# Autodesk Inventor assembly: HACKberry_v1_for_print_Hand_withCaseC
Saved by Autodesk Inventor 2016 (Build 200138000, 138)
## iProperties
Created: 2016-06-07
Part Number: HACKberry_v1_for_print_Hand_withCaseC
Material: 一般
Document SubType Name: Assembly
Designer: Yamaura
Author: Yamaura
## Documents named in this file (9)
- C:\Users\Yamaura\Documents\GitHub\HACKberry\HACKberry-hardware\3D\Inventor\Parts\HACKberry_v1_for_print_Hand_withCaseC.iam
- C:\Users\Yamaura\Documents\GitHub\HACKberry\HACKberry-hardware\3D\Inventor\Parts\HbBatteryCase01.ipt
- C:\Users\Yamaura\Documents\GitHub\HACKberry\HACKberry-hardware\3D\Inventor\Parts\HbMiddle-DistalPhalanx02.ipt
- C:\Users\Yamaura\Documents\GitHub\HACKberry\HACKberry-hardware\3D\Inventor\Parts\HbProximalPhalanx02.ipt
- C:\Users\Yamaura\Documents\GitHub\HACKberry\HACKberry-hardware\3D\Inventor\Parts\HbProximalPhalanxCover02.ipt
- C:\Users\Yamaura\Documents\GitHub\HACKberry\HACKberry-hardware\3D\Inventor\Parts\HbCouplerLink02.ipt
- C:\Users\Yamaura\Documents\GitHub\HACKberry\HACKberry-hardware\3D\Inventor\Parts\HbCouplerLinkCover03.ipt
- C:\Users\Yamaura\Documents\GitHub\HACKberry\HACKberry-hardware\3D\Inventor\Parts\HbShaftStopperB04.ipt
- C:\Users\Yamaura\Documents\GitHub\HACKberry\HACKberry-hardware\3D\Inventor\Parts\HbShaftStopperA04.ipt
## Components (10 placed, 8 different names)
1. HbBatteryCase01:1
2. HbMiddle-DistalPhalanx02_1
3. HbProximalPhalanx02_1
4. HbProximalPhalanxCover02_1
5. HbCouplerLink02_1
6. HbCouplerLinkCover03_1
7. HbShaftStopperB04:1
8. HbShaftStopperB04:2
9. HbShaftStopperA04:1
10. HbShaftStopperA04:2
## Component patterns: (2 elements, first: HbShaftStopperB04:1), (2 elements, first: HbShaftStopperA04:1)
